# Autodesk Inventor assembly: 3 Postion Pneumatic Cylinder (9-16 in Bore, .25 in ,2 in stroke)
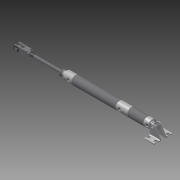
[picture p0: Inventor's stored thumbnail of the model, 180x180]
Saved by Autodesk Inventor 2014 (Build 180170000, 170)
## iProperties
Category: PARTsolutions
Company: BIMBA
Created: 2014-01-22
Part Number: 3 Postion Pneumatic Cylinder (9-16 in Bore, .25 in ,2 in stroke)
Catalog Web Link: www.cadenas.de
Description: Original Line Three-Position Cylinders-
Vendor: BIMBA
Document SubType Name: Assembly
Designer: Michael
Manufacturer: BIMBA
PSOL_IDENT_0: {$CADENAS_DATA\23d-libs\bimba\bimba\bimba_imperial\bimba_full_line\original_line_cylinders\three_pos
PSOL_IDENT_1: ition_cylinders\3position_asmtab.prj},292 {VTYP=3D},{STYP=ASSTAB},{NB=020.25/2-DXP(D-850)(D-12321-A)
PSOL_IDENT_2: },{LINA=020.25/2-DXP},{NN=Original Line Three-Position Cylinders},{DATE=15.10.2013 05:44:09},{GEOMDA
PSOL_IDENT_3: TE=27.08.2012},{VERSION=},{LINEID=40},{LINESUBID=-1},{WBVAR=STROKEA,STROKEB,MNT,NR,M,NT,EE,EEL,G,K,Q
PSOL_IDENT_4: ,B,T,W,T1,T2,T3,T4,PRC,MB,MN,PB}  {NB=020.25/2-DXP(D-850)(D-12321-A)},{LINA=020.25/2-DXP},{KT=DUMMY}
PSOL_IDENT_5: ,{PN=020.25/2-DXP},{PNC=020.25/2-DXP(D-850)(D-12321-A)},{PNA=(D-850)(D-12321-A)},{DASH=-},{BORE1=0.5
PSOL_IDENT_6: 6250000},{BORE=9/16\" (02)},{BOREPN=02},{STROKEA=0.250},{STROKEB=2.000},{STROKEALGA=[0.011:31.989/0.
PSOL_IDENT_7: 001]},{STROKEALGB=[0.011:31.75/0.001]},{STROKEBMAX=31.75},{STROKE1=0.25},{STROKE2=2.000},{AC=Double
PSOL_IDENT_8: Acting},{ACTING=D},{ACTINGALG= 'D' , 'Double Acting' },{ACTINGPN=D},{MNT=XP},{MNTALG= '' , 'Nose Mou
PSOL_IDENT_9: nting (3P)' , 'XP' , 'Universal Mounting (3P)' },{MNTPN=XP},{TYPE=},{NR=},{NRALG= '' , 'Round (Stand
PSOL_IDENT_10: ard)' , 'NR' , 'Non-Rotating Square' },{NRPN=},{M=},{MALG= '', 'Without Magnet', 'M', 'With Magnet'
PSOL_IDENT_11: },{MATR=303 Stainless Steel},{F=},{FALG= '', 'Non-Coated (Standard)', 'F', 'Molycoated' },{FPN=},{NT=
PSOL_IDENT_12: },{NTPN=},{EE=},{EEL=0.000},{EEMAX=29.750},{EEALG= '', 'Without Extra Extension', 'EE', 'With Extra
PSOL_IDENT_13: Extension' },{EELALG=0},{EEPN=},{EEPN1=0.000},{G=},{GPN=},{GPN1=},{K=},{KALG= '', 'Standard' , 'K' ,
PSOL_IDENT_14: 'Ports Rotated 90deg K' },{KPN=},{Q=},{QALG= '' , 'N/A' },{QPN=},{B=},{BALG= '', 'Without Bumper' ,
PSOL_IDENT_15: 'B' , 'With Bumper' },{BPN=},{T=},{TALG= '' , 'Standard -20° to 200°F (-29° to 95°C)' , 'N' , 'Low
PSOL_IDENT_16: Temperature' , 'V' , 'High Temperature' },{NPN=},{VPN=},{W=},{WALG= '' , 'Without Wiper' , 'W' , 'Wi
PSOL_IDENT_17: th Wiper' },{WPN=},{E=},{EALG= '' , 'Standard Seals/Lube' , 'E' , 'Non-Lube Seals/Lube' },{EPN=},{ST=
PSOL_IDENT_18: },{STALG= '' , 'Without Switch Track' , '-' , 'With Switch Track' },{STPALG= '' , 'N/A' },{STPN=},{T
PSOL_IDENT_19: 1=},{T2=},{T3=},{T4=},{S=},{SALG='','N/A'},{SPN=},{PRC=D-850},{PRCALG= '' , 'w/out Pivot Rod Clevis'
PSOL_IDENT_20: , 'D-850' , 'D-850'},{PRCPN=(D-850)},{MB=},{MN=},{PB=D-12321-A},{PBALG= '' , 'w/out Pivot Bracket'
PSOL_IDENT_21: , 'D-12321-A' , 'D-12321-A' },{PBPN=(D-12321-A)},{TLEN=1.757},{TEXT=0.116667},{SPACE=0.066667},{FRAC=
PSOL_IDENT_22: 3.97},{BL=},{BR=},{DWGC=},{PNN=},{MNTRG=},{ACTINGRG=R},{DIMBRL=2.28100000},{DIMBRE=1.65600000},{DIMB
PSOL_IDENT_23: BL=1.00000000},{RLB=4.531},{REB=3.906},{BLB=3.250},{DIMARL=1.85600000},{DIMARE=1.23100000},{DIMABL=0
PSOL_IDENT_24: .93800000},{RLA=2.106},{REA=1.481},{BLA=1.188},{DWGCS=D-68355},{DWGTA=D-75938},{DWGTB=D-7516},{DWGRH=
PSOL_IDENT_25: D-15705},{DWGRG=D-26368},{TRANS=0.50000000},{DWGRCB=D-7508},{DWGRCA=D-9538},{BRL=2.50000000},{BRE=1.
PSOL_IDENT_26: 57800000},{BBL=1.06200000},{ARL=1.91600000},{ARE=0.99400000},{ABL=1.06200000},{T1ALG='','N/A'},{T2AL
PSOL_IDENT_27: G='','N/A'},{T3ALG='','N/A'},{T4ALG='','N/A'},{DWGST=D-74168},{DWGS=},{STL=2.9},{TS=X},{SS=},{AA=4.4
PSOL_IDENT_28: 0},{BA=2.25},{C=0.75},{D=#10-32},{E1=0.38},{E11=0.38000000},{E12=0.38000000},{F1=0.06},{G1=N/A},{H=0
PSOL_IDENT_29: .50},{I=7/16-20},{J=N/A},{K1=#10-32},{L1=.434/.437},{M1=0.38},{N=0.31},{O=0.62},{AA1=4.12000000},{BA
PSOL_IDENT_30: 1=2.25000000},{AA1B=4.31000000},{BA1B=2.31000000},{AA1XP=4.40000000},{BA1XP=2.25000000},{AA1BXP=4.59
PSOL_IDENT_31: 000000},{BA1BXP=2.31000000},{M11=0.19000000},{M12=0.38000000},{N1=0.50000000},{N2=0.31000000},{O1=0.
PSOL_IDENT_32: 62000000},{O2=0.62000000},{P=0.25},{Q1=0.19},{R=0.16},{P1=0.25000000},{Q11=0.19000000},{R1=0.16},{MB
PSOL_IDENT_33: ALG= '' , 'w/out Mounting Bracket' , 'F,D-770' , 'D-770 (front)', 'R,D-770' , 'D-770 (rear)', '2x,D-
PSOL_IDENT_34: 770' , 'D-770 (front & rear)' },{MBPN=},{MBP=},{MNALG= '' , 'w/out Mounting Nut' , 'F,D-154' , 'D-15
PSOL_IDENT_35: 4 (front)', 'R,D-154' , 'D-154 (rear)', '2x,D-154' , 'D-154 (front & rear)' },{MNPN=},{MNP=},{PRCP=}
PSOL_IDENT_36: ,{MBR=},{MBF=},{MNF=},{MNR=},{PBPNALL=D-12321-A},{MBPNALL=D-770},{PRCPNALL=D-850},{FNUTPN=D-154},{RN
PSOL_IDENT_37: UTPN=D-154},{ASSOPTACC=T4},{MATALGHTML=<b>Original Line Three Position:</b><dl><dt>Rod:</dt><dd>- 30
PSOL_IDENT_38: 3 Stainless Steel</dd><dt>Bearings:</dt><dd>- Sintered Bronze</dd><dt>Body:</dt><dd>- 304 Stainless
PSOL_IDENT_39: Steel</dd><dt>End Caps:</dt><dd>- Aluminum</dd><dt>Seals:</dt><dd>-  Buna N</dd></dl>},{PPATH=three_
PSOL_IDENT_40: pos_cylinder_asmtpl.prj}
CNS_NN: Original Line Three-Position Cylinders
CNS_NT: Standard Male Thread
CNS_NB: 020.25/2-DXP(D-850)(D-12321-A)
CNS_NBSYN: $PNC.
CNS_LINA: 020.25/2-DXP
CNS_PN: 020.25/2-DXP
CNS_PNC: 020.25/2-DXP(D-850)(D-12321-A)
CNS_PNA: (D-850)(D-12321-A)
CNS_DASH: -
CNS_BORE1: 0.56250000
CNS_BORE: 9/16" [02]
CNS_BOREPN: 02
CNS_STROKEA: 0.250
CNS_STROKEB: 2.000
CNS_STROKEALGA: [0.011:31.989/0.001]
CNS_STROKEALGB: [0.011:31.75/0.001]
CNS_STROKEBMAX: 31.750
CNS_STROKE1: 0.250
CNS_STROKE2: 2.000
CNS_AC: Double
CNS_ACTING: D
CNS_ACTINGALG: 'D' , 'Double Acting'
CNS_ACTINGPN: D
CNS_MNT: Universal Double End or Rear Pivot [DXP]
CNS_MNTALG: '' , 'Nose Mounting (3P)' , 'XP' , 'Universal Mounting (3P)'
CNS_MNTPN: XP
CNS_NR: Standard Round
CNS_NRALG: '' , 'Round (Standard)' , 'NR' , 'Non-Rotating Square'
CNS_M: Without Magnet Piston
CNS_MALG: '', 'Without Magnet', 'M', 'With Magnet'
CNS_MATR: Stainless Steel
CNS_FALG: '', 'Non-Coated (Standard)', 'F', 'Molycoated'
CNS_EE: Standard Rod Extension
CNS_EEL: 0.000
CNS_EEMAX: 29.750
CNS_EEALG: '', 'Without Extra Extension', 'EE', 'With Extra Extension'
CNS_EELALG: 0
CNS_EEPN1: 0.000
CNS_G: Standard Grease Lube
CNS_K: Standard
CNS_KALG: '', 'Standard' , 'K' , 'Ports Rotated 90deg K'
CNS_Q: N/A
CNS_QALG: '' , 'N/A'
CNS_B: Without Bumpers
CNS_BALG: '', 'Without Bumper' , 'B' , 'With Bumper'
CNS_T: Standard -20° to 200°F (-29° to 95°C)
CNS_TALG: '' , 'Standard -20° to 200°F (-29° to 95°C)' , 'N' , 'Low Temperature' , 'V' , 'High Temperature'
CNS_W: Without Wiper
CNS_WALG: '' , 'Without Wiper' , 'W' , 'With Wiper'
CNS_EALG: '' , 'Standard Seals/Lube' , 'E' , 'Non-Lube Seals/Lube'
CNS_STALG: '' , 'Without Switch Track' , '-' , 'With Switch Track'
CNS_STPALG: '' , 'N/A'
CNS_T1: N/A
CNS_T2: N/A
CNS_T3: N/A
CNS_T4: N/A
CNS_SALG: '','N/A'
CNS_PRC: D-850
CNS_PRCALG: '' , 'w/out Pivot Rod Clevis' , 'D-850' , 'D-850'
CNS_PRCPN: (D-850)
CNS_MB: Without Mounting Bracket
CNS_MN: Without Mounting Nut
CNS_PB: D-12321-A
CNS_PBALG: '' , 'w/out Pivot Bracket' , 'D-12321-A' , 'D-12321-A'
CNS_PBPN: (D-12321-A)
CNS_TLEN: 1.757
CNS_TEXT: 0.117
CNS_SPACE: 0.067
CNS_FRAC: 3.970
CNS_ACTINGRG: R
CNS_DIMBRL: 2.28100000
CNS_DIMBRE: 1.65600000
CNS_DIMBBL: 1.00000000
CNS_RLB: 4.531
CNS_REB: 3.906
CNS_BLB: 3.250
CNS_DIMARL: 1.85600000
CNS_DIMARE: 1.23100000
CNS_DIMABL: 0.93800000
CNS_RLA: 2.106
CNS_REA: 1.481
CNS_BLA: 1.188
CNS_DWGCS: D-68355
CNS_DWGTA: D-75938
CNS_DWGTB: D-7516
CNS_DWGRH: D-15705
CNS_DWGRG: D-26368
CNS_TRANS: 0.50000000
CNS_DWGRCB: D-7508
CNS_DWGRCA: D-9538
CNS_BRL: 2.50000000
CNS_BRE: 1.57800000
CNS_BBL: 1.06200000
CNS_ARL: 1.91600000
CNS_ARE: 0.99400000
CNS_ABL: 1.06200000
CNS_T1ALG: '','N/A'
CNS_T2ALG: '','N/A'
CNS_T3ALG: '','N/A'
CNS_T4ALG: '','N/A'
CNS_DWGST: D-74168
CNS_STL: 2.900
CNS_TS: X
CNS_AA: 4.40
CNS_BA: 2.25
CNS_C: 0.75
CNS_D: #10-32
CNS_E1: 0.38
CNS_E11: 0.38000000
CNS_E12: 0.38000000
CNS_F1: 0.06
CNS_G1: N/A
CNS_H: 0.50
CNS_I: 7/16-20
CNS_J: N/A
CNS_K1: #10-32
CNS_L1: .434/.437
CNS_M1: 0.38
CNS_N: 0.31
CNS_O: 0.62
CNS_AA1: 4.12000000
CNS_BA1: 2.25000000
CNS_AA1B: 4.31000000
CNS_BA1B: 2.31000000
CNS_AA1XP: 4.40000000
CNS_BA1XP: 2.25000000
CNS_AA1BXP: 4.59000000
CNS_BA1BXP: 2.31000000
CNS_M11: 0.19000000
CNS_M12: 0.38000000
CNS_N1: 0.50000000
CNS_N2: 0.31000000
CNS_O1: 0.62000000
CNS_O2: 0.62000000
CNS_P: 0.25
CNS_Q1: 0.19
CNS_R: 0.16
CNS_P1: 0.25000000
CNS_Q11: 0.19000000
CNS_R1: 0.16
CNS_MBALG: '' , 'w/out Mounting Bracket' , 'F,D-770' , 'D-770 (front)', 'R,D-770' , 'D-770 (rear)', '2x,D-770' , 'D-770 (front & rear)'
CNS_MNALG: '' , 'w/out Mounting Nut' , 'F,D-154' , 'D-154 (front)', 'R,D-154' , 'D-154 (rear)', '2x,D-154' , 'D-154 (front & rear)'
CNS_PBPNALL: D-12321-A
CNS_MBPNALL: D-770
CNS_PRCPNALL: D-850
CNS_FNUTPN: D-154
CNS_RNUTPN: D-154
CNS_ASSOPTACC: T4
CNS_MATALGHTML: <b>Original Line Three Position:</b><dl><dt>Rod:</dt><dd>- 303 Stainless Steel</dd><dt>Bearings:</dt><dd>- Sintered Bronze</dd><dt>Body:</dt><dd>- 304 Stainless Steel</dd><dt>End Caps:</dt><dd>- Aluminum</dd><dt>Seals:</dt><dd>-  Buna N</dd></dl>
CNS_PPATH: three_pos_cylinder_asmtpl.prj
SUPPLIER: BIMBA
ARTICLENO: 020.25/2-DXP(D-850)(D-12321-A)
BOMINFO: 020.25/2-DXP
CREATOR: CADENAS GmbH
Title: 020.25/2-DXP
Author: Cadenas PARTsolutions
## Documents named in this file (20)
- C:\Users\Michael\Documents\GitHub\2014buildCAD\New Collector\3 Postion Pneumatic Cylinder (9-16 in Bore, .25 in ,2 in stroke).iam
- C:\Users\Michael\Documents\GitHub\2014buildCAD\New Collector\020_25_2-DXP(D-850)(D-12321-A)0_dummy.ipt
- C:\Users\Michael\Documents\GitHub\2014buildCAD\New Collector\D-68355-XP--0.ipt
- C:\Users\Michael\Documents\GitHub\2014buildCAD\New Collector\D-75938XP-1_188.ipt
- C:\Users\Michael\Documents\GitHub\2014buildCAD\New Collector\D-15705rear_head.ipt
- C:\Users\Michael\Documents\GitHub\2014buildCAD\New Collector\D-8597.ipt
- C:\Users\Michael\Documents\GitHub\2014buildCAD\New Collector\D-12321-A-dummy.ipt
- C:\Users\Michael\Documents\GitHub\2014buildCAD\New Collector\D-9963_pin.ipt
- C:\Users\Michael\Documents\GitHub\2014buildCAD\New Collector\D-782_pin.ipt
- C:\Users\Michael\Documents\GitHub\2014buildCAD\New Collector\D-9769-clevis_pin.ipt
- C:\Users\Michael\Documents\GitHub\2014buildCAD\New Collector\D-9770-rr.ipt
- C:\Users\Michael\Documents\GitHub\2014buildCAD\New Collector\D-7516XP-3_25.ipt
- C:\Users\Michael\Documents\GitHub\2014buildCAD\New Collector\D-26368----0_5_rod_guide_cyl.ipt
- C:\Users\Michael\Documents\GitHub\2014buildCAD\New Collector\D-75080_25-2XP-4_531-3pos.ipt
- C:\Users\Michael\Documents\GitHub\2014buildCAD\New Collector\D-850-dummy.ipt
- C:\Users\Michael\Documents\GitHub\2014buildCAD\New Collector\D-14043.ipt
- C:\Users\Michael\Documents\GitHub\2014buildCAD\New Collector\D-12304.ipt
- C:\Users\Michael\Documents\GitHub\2014buildCAD\New Collector\D-5406.ipt
- C:\Users\Michael\Documents\GitHub\2014buildCAD\New Collector\D-5288.ipt
- C:\Users\Michael\Documents\GitHub\2014buildCAD\New Collector\D-95380_25-2XP-2_106-3pos.ipt
## Components (21 placed, 19 different names)
1. 020_25_2-DXP(D-850)(D-12321-A)0_dummy:1 — dummy_XY@1 <-> centar_XY@2, dummy_Z@1 <-> centar_Z@2, dummy_YZ@1 <-> centar_YZ@2
2. D-68355-XP--0:1 — dummy_XY@1 <-> centar_XY@2, dummy_Z@1 <-> centar_Z@2, dummy_YZ@1 <-> centar_YZ@2, to_cyl_A_XY@2 <-> tube2_XY@3, to_cyl_A_Z@2 <-> tube2_Z@3, to_cyl_A_YZ@2 <-> tube2_YZ@3, to_cyl_B_XY@2 <-> tube1_XY@12, to_cyl_B_Z@2 <-> tube1_Z@12, to_cyl_B_YZ@2 <-> tube1_YZ@12, to_rod_A_XY@2 <-> to_rod_guide_XY@21, to_rod_A_Z@2 <-> to_rod_guide_Z@21
3. D-75938XP-1_188:1 — to_cyl_A_XY@2 <-> tube2_XY@3, to_cyl_A_Z@2 <-> tube2_Z@3, to_cyl_A_YZ@2 <-> tube2_YZ@3, tube1_XY@3 <-> rear_head_XY@4, tube1_Z@3 <-> rear_head_Z@4, tube1_YZ@3 <-> rear_head_YZ@4
4. D-15705rear_head:1 — tube1_XY@3 <-> rear_head_XY@4, tube1_Z@3 <-> rear_head_Z@4, tube1_YZ@3 <-> rear_head_YZ@4, to_bushing_XY@4 <-> bushing_XY@5, to_bushing_Z@4 <-> bushing_Z@5, to_bushing_YZ@4 <-> bushing_YZ@5, to_pivot_bracket_XY@4 <-> to_cyl_XY@6, to_pivot_bracket_Z@4 <-> to_cyl_Z@6
5. D-8597:1 — to_bushing_XY@4 <-> bushing_XY@5, to_bushing_Z@4 <-> bushing_Z@5, to_bushing_YZ@4 <-> bushing_YZ@5
6. D-12321-A-dummy:1 — to_pivot_bracket_XY@4 <-> to_cyl_XY@6, to_pivot_bracket_Z@4 <-> to_cyl_Z@6, to_l_XY@6 <-> to_dummy_L_XY@7, to_l_Z@6 <-> to_dummy_L_Z@7, to_l_YZ@6 <-> to_dummy_L_YZ@7, to_r_XY@6 <-> to_dummy_R_XY@8, to_r_Z@6 <-> to_dummy_R_Z@8, to_r_YZ@6 <-> to_dummy_R_YZ@8
7. D-9963_pin:1 — to_l_XY@6 <-> to_dummy_L_XY@7, to_l_Z@6 <-> to_dummy_L_Z@7, to_l_YZ@6 <-> to_dummy_L_YZ@7
8. D-782_pin:1 — to_r_XY@6 <-> to_dummy_R_XY@8, to_r_Z@6 <-> to_dummy_R_Z@8, to_r_YZ@6 <-> to_dummy_R_YZ@8, to_pin_R_XY@8 <-> pin_XY@9, to_pin_R_Z@8 <-> pin_Z@9, to_pin_R_YZ@8 <-> pin_YZ@9
9. D-9769-clevis_pin:1 — to_pin_R_XY@8 <-> pin_XY@9, to_pin_R_Z@8 <-> pin_Z@9, to_pin_R_YZ@8 <-> pin_YZ@9, rr1_XY@9 <-> rr_XY@10, rr1_Z@9 <-> rr_Z@10, rr1_YZ@9 <-> rr_YZ@10, rr2_XY@9 <-> rr_XY@11, rr2_Z@9 <-> rr_Z@11, rr2_YZ@9 <-> rr_YZ@11
10. D-9770-rr:1 — rr1_XY@9 <-> rr_XY@10, rr1_Z@9 <-> rr_Z@10, rr1_YZ@9 <-> rr_YZ@10
11. D-9770-rr:2 — rr2_XY@9 <-> rr_XY@11, rr2_Z@9 <-> rr_Z@11, rr2_YZ@9 <-> rr_YZ@11
12. D-7516XP-3_25:1 — to_cyl_B_XY@2 <-> tube1_XY@12, to_cyl_B_Z@2 <-> tube1_Z@12, to_cyl_B_YZ@2 <-> tube1_YZ@12, tube2_XY@12 <-> to_tube_XY@13, tube2_Z@12 <-> to_tube_Z@13, tube2_YZ@12 <-> to_tube_YZ@13
13. D-26368----0_5_rod_guide_cyl:1 — tube2_XY@12 <-> to_tube_XY@13, tube2_Z@12 <-> to_tube_Z@13, tube2_YZ@12 <-> to_tube_YZ@13, to_rod_XY@13 <-> to_rod_guide_XY@14, to_rod_Z@13 <-> to_rod_guide_Z@14, Flush:7
14. D-75080_25-2XP-4_531-3pos:1 — to_rod_XY@13 <-> to_rod_guide_XY@14, to_rod_Z@13 <-> to_rod_guide_Z@14, to_rod_guide_XY@14 <-> from_prc_XY@15, to_rod_guide_Z@14 <-> from_prc_Z@15, Flush:7
15. D-850-dummy:1 — to_rod_guide_XY@14 <-> from_prc_XY@15, to_rod_guide_Z@14 <-> from_prc_Z@15, dummy_XY@15 <-> dummy_XY@16, dummy_Z@15 <-> dummy_Z@16, dummy_YZ@15 <-> dummy_YZ@16
16. D-14043:1 — dummy_XY@15 <-> dummy_XY@16, dummy_Z@15 <-> dummy_Z@16, dummy_YZ@15 <-> dummy_YZ@16, rod_clevis_body_XY@16 <-> pin_XY@17, rod_clevis_body_Z@16 <-> pin_Z@17, piston_rod_clevis_XY@16 <-> NUT_XY@20, piston_rod_clevis_Z@16 <-> NUT_Z@20
17. D-12304:1 — rod_clevis_body_XY@16 <-> pin_XY@17, rod_clevis_body_Z@16 <-> pin_Z@17, rr1_XY@17 <-> RR_XY@18, rr1_Z@17 <-> RR_Z@18, rr2_XY@17 <-> RR_XY@19, rr2_Z@17 <-> RR_Z@19
18. D-5406:1 — rr1_XY@17 <-> RR_XY@18, rr1_Z@17 <-> RR_Z@18
19. D-5406:2 — rr2_XY@17 <-> RR_XY@19, rr2_Z@17 <-> RR_Z@19
20. D-5288:1 — piston_rod_clevis_XY@16 <-> NUT_XY@20, piston_rod_clevis_Z@16 <-> NUT_Z@20
21. D-95380_25-2XP-2_106-3pos:1 — to_rod_A_XY@2 <-> to_rod_guide_XY@21, to_rod_A_Z@2 <-> to_rod_guide_Z@21
## Relationships (53: Mate 34, Angle 12, Flush 7)
- dummy_XY@1 <-> centar_XY@2 [Mate]: 020_25_2-DXP(D-850)(D-12321-A)0_dummy:1 ↔ D-68355-XP--0:1
- dummy_Z@1 <-> centar_Z@2 [Mate]: 020_25_2-DXP(D-850)(D-12321-A)0_dummy:1 ↔ D-68355-XP--0:1
- dummy_YZ@1 <-> centar_YZ@2 [Angle] (-90 deg): 020_25_2-DXP(D-850)(D-12321-A)0_dummy:1 ↔ D-68355-XP--0:1
- to_cyl_A_XY@2 <-> tube2_XY@3 [Flush]: D-68355-XP--0:1 ↔ D-75938XP-1_188:1
- to_cyl_A_Z@2 <-> tube2_Z@3 [Mate]: D-68355-XP--0:1 ↔ D-75938XP-1_188:1
- to_cyl_A_YZ@2 <-> tube2_YZ@3 [Angle] (0 deg): D-68355-XP--0:1 ↔ D-75938XP-1_188:1
- tube1_XY@3 <-> rear_head_XY@4 [Mate]: D-75938XP-1_188:1 ↔ D-15705rear_head:1
- tube1_Z@3 <-> rear_head_Z@4 [Mate]: D-75938XP-1_188:1 ↔ D-15705rear_head:1
- tube1_YZ@3 <-> rear_head_YZ@4 [Angle] (90 deg): D-75938XP-1_188:1 ↔ D-15705rear_head:1
- to_bushing_XY@4 <-> bushing_XY@5 [Mate]: D-15705rear_head:1 ↔ D-8597:1
- to_bushing_Z@4 <-> bushing_Z@5 [Mate]: D-15705rear_head:1 ↔ D-8597:1
- to_bushing_YZ@4 <-> bushing_YZ@5 [Angle] (0 deg): D-15705rear_head:1 ↔ D-8597:1
- to_pivot_bracket_XY@4 <-> to_cyl_XY@6 [Mate]: D-15705rear_head:1 ↔ D-12321-A-dummy:1
- to_pivot_bracket_Z@4 <-> to_cyl_Z@6 [Mate]: D-15705rear_head:1 ↔ D-12321-A-dummy:1
- to_l_XY@6 <-> to_dummy_L_XY@7 [Flush]: D-12321-A-dummy:1 ↔ D-9963_pin:1
- to_l_Z@6 <-> to_dummy_L_Z@7 [Mate]: D-12321-A-dummy:1 ↔ D-9963_pin:1
- to_l_YZ@6 <-> to_dummy_L_YZ@7 [Angle] (0 deg): D-12321-A-dummy:1 ↔ D-9963_pin:1
- to_r_XY@6 <-> to_dummy_R_XY@8 [Flush]: D-12321-A-dummy:1 ↔ D-782_pin:1
- to_r_Z@6 <-> to_dummy_R_Z@8 [Mate]: D-12321-A-dummy:1 ↔ D-782_pin:1
- to_r_YZ@6 <-> to_dummy_R_YZ@8 [Angle] (0 deg): D-12321-A-dummy:1 ↔ D-782_pin:1
- to_pin_R_XY@8 <-> pin_XY@9 [Mate] (4.191 mm): D-782_pin:1 ↔ D-9769-clevis_pin:1
- to_pin_R_Z@8 <-> pin_Z@9 [Mate]: D-782_pin:1 ↔ D-9769-clevis_pin:1
- to_pin_R_YZ@8 <-> pin_YZ@9 [Angle] (0 deg): D-782_pin:1 ↔ D-9769-clevis_pin:1
- rr1_XY@9 <-> rr_XY@10 [Mate]: D-9769-clevis_pin:1 ↔ D-9770-rr:1
- rr1_Z@9 <-> rr_Z@10 [Mate]: D-9769-clevis_pin:1 ↔ D-9770-rr:1
- rr1_YZ@9 <-> rr_YZ@10 [Angle] (0 deg): D-9769-clevis_pin:1 ↔ D-9770-rr:1
- rr2_XY@9 <-> rr_XY@11 [Mate]: D-9769-clevis_pin:1 ↔ D-9770-rr:2
- rr2_Z@9 <-> rr_Z@11 [Mate]: D-9769-clevis_pin:1 ↔ D-9770-rr:2
- rr2_YZ@9 <-> rr_YZ@11 [Angle] (0 deg): D-9769-clevis_pin:1 ↔ D-9770-rr:2
- to_cyl_B_XY@2 <-> tube1_XY@12 [Flush]: D-68355-XP--0:1 ↔ D-7516XP-3_25:1
- to_cyl_B_Z@2 <-> tube1_Z@12 [Mate]: D-68355-XP--0:1 ↔ D-7516XP-3_25:1
- to_cyl_B_YZ@2 <-> tube1_YZ@12 [Angle] (0 deg): D-68355-XP--0:1 ↔ D-7516XP-3_25:1
- tube2_XY@12 <-> to_tube_XY@13 [Mate]: D-7516XP-3_25:1 ↔ D-26368----0_5_rod_guide_cyl:1
- tube2_Z@12 <-> to_tube_Z@13 [Mate]: D-7516XP-3_25:1 ↔ D-26368----0_5_rod_guide_cyl:1
- tube2_YZ@12 <-> to_tube_YZ@13 [Angle] (-180 deg): D-7516XP-3_25:1 ↔ D-26368----0_5_rod_guide_cyl:1
- to_rod_XY@13 <-> to_rod_guide_XY@14 [Flush]: D-26368----0_5_rod_guide_cyl:1 ↔ D-75080_25-2XP-4_531-3pos:1
- to_rod_Z@13 <-> to_rod_guide_Z@14 [Mate]: D-26368----0_5_rod_guide_cyl:1 ↔ D-75080_25-2XP-4_531-3pos:1
- to_rod_guide_XY@14 <-> from_prc_XY@15 [Flush]: D-75080_25-2XP-4_531-3pos:1 ↔ D-850-dummy:1
- to_rod_guide_Z@14 <-> from_prc_Z@15 [Mate]: D-75080_25-2XP-4_531-3pos:1 ↔ D-850-dummy:1
- dummy_XY@15 <-> dummy_XY@16 [Mate]: D-850-dummy:1 ↔ D-14043:1
- dummy_Z@15 <-> dummy_Z@16 [Mate]: D-850-dummy:1 ↔ D-14043:1
- dummy_YZ@15 <-> dummy_YZ@16 [Angle] (0 deg): D-850-dummy:1 ↔ D-14043:1
- rod_clevis_body_XY@16 <-> pin_XY@17 [Mate]: D-14043:1 ↔ D-12304:1
- rod_clevis_body_Z@16 <-> pin_Z@17 [Mate]: D-14043:1 ↔ D-12304:1
- rr1_XY@17 <-> RR_XY@18 [Mate]: D-12304:1 ↔ D-5406:1
- rr1_Z@17 <-> RR_Z@18 [Mate]: D-12304:1 ↔ D-5406:1
- rr2_XY@17 <-> RR_XY@19 [Mate]: D-12304:1 ↔ D-5406:2
- rr2_Z@17 <-> RR_Z@19 [Mate]: D-12304:1 ↔ D-5406:2
- piston_rod_clevis_XY@16 <-> NUT_XY@20 [Mate]: D-14043:1 ↔ D-5288:1
- piston_rod_clevis_Z@16 <-> NUT_Z@20 [Mate]: D-14043:1 ↔ D-5288:1
- to_rod_A_XY@2 <-> to_rod_guide_XY@21 [Mate]: D-68355-XP--0:1 ↔ D-95380_25-2XP-2_106-3pos:1
- to_rod_A_Z@2 <-> to_rod_guide_Z@21 [Mate]: D-68355-XP--0:1 ↔ D-95380_25-2XP-2_106-3pos:1
- Flush:7 (-50.8 mm): D-26368----0_5_rod_guide_cyl:1 ↔ D-75080_25-2XP-4_531-3pos:1
